# Autodesk Inventor assembly: KTN_MultiPass
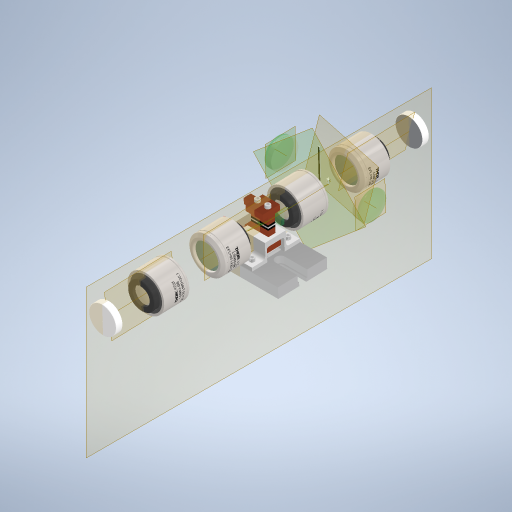
[picture p0: Inventor's stored thumbnail of the model, 512x512]
Saved by Autodesk Inventor 2023 (Build 270158000, 158)
## iProperties
Created: 2024-04-24
Part Number: KTN_MultiPass
Document SubType Name: Assembly
Designer: kerlin
Author: kerlin
## iProperties of the stored document base_Al_LEOD.ipt
Created: 2023-03-07
Part Number: bottomblock_al_ledgereod
Material: Aluminum 6061
Document SubType Name: Modeling
Designer: warke
Density: 2.7 g/cm^3
Appearance: Default
Sending System: Autodesk Inventor 2024
Author: warke
## iProperties of the stored document KTN_Chip_6p6mm_4mm_1p2mm_WithElectrodes.ipt
Created: 2022-10-15
Part Number: KTN_Chip_6p6mm_4mm_1p2mm_WithElectrodes
Material: Generic
Document SubType Name: Modeling
Designer: kerlin
Density: 1 g/cm^3
Appearance: Default
Sending System: Autodesk Inventor 2024
Author: kerlin
## iProperties of the stored document TEC3-2.5-Solidworks (1).ipt
Created: 2005-09-14
Part Number: TEC3-2.5-Solidworks (1)
Material: Generic
Document SubType Name: Modeling
Designer: warke
Density: 1 g/cm^3
Appearance: Default
Sending System: SolidWorks 2005
Last Author: rsavioli
Last Saved: 2005-09-14
Author: warke
## iProperties of the stored document 92196A107_18-8 Stainless Steel Socket Head Screw.ipt
Created: 2021-02-02
Part Number: 92196A107
Material: Generic
Description: 18-8 Stainless Steel Socket Head Screw
Vendor: McMaster-Carr Supply Company
Document SubType Name: Modeling
Designer: warke
Density: 1 g/cm^3
Appearance: Default
Sending System: SolidWorks 2017
Last Author: intuser33
Last Saved: 2023-02-03
Material: 18-8 Stainless Steel
Copyright: © 2023 McMaster-Carr Supply Company
CAD Model Disclaimer and Terms of Use: https://www.mcmaster.com/terms
Desc1: 18-8 Stainless Steel
Desc2: Socket Head Screw
Desc3: © 2023 McMaster-Carr Supply Company
Author: warke
## iProperties of the stored document spacer_AlN_LEOD.ipt
Created: 2023-03-13
Part Number: shapal_ledgereod
Material: Generic
Document SubType Name: Modeling
Designer: warke
Density: 1 g/cm^3
Appearance: Default
Sending System: Autodesk Inventor 2024
Author: warke
## iProperties of the stored document peltierclip_LEOD.ipt
Created: 2023-03-14
Part Number: peltierclip_ledgereod2
Material: Generic
Document SubType Name: Modeling
Designer: warke
Density: 1 g/cm^3
Appearance: Default
Sending System: Autodesk Inventor 2024
Author: warke
## iProperties of the stored document EOD_D1_v2.0.iam
Created: 2023-03-15
Part Number: EOD_D1_v2.0
Document SubType Name: Assembly
Designer: warke
Sending System: Autodesk Inventor 2024
Author: warke
## iProperties of the stored document 92949A105_18-8 Stainless Steel Button Head Hex Drive Screw.ipt
Created: 2019-06-06
Part Number: 92949A105_18-8 Stainless Steel Button Head Hex Drive Screw
Material: Stainless Steel, Austenitic
Description: 18-8 Stainless Steel Button Head Hex Drive Screw
Vendor: McMaster-Carr Supply Company
Document SubType Name: Modeling
Designer: warke
Density: 8 g/cm^3
Appearance: Default
Sending System: SolidWorks 2017
Last Author: intuser33
Last Saved: 2022-09-28
Material: 18-8 Stainless Steel
Copyright: © 2022 McMaster-Carr Supply Company
CAD Model Disclaimer and Terms of Use: https://www.mcmaster.com/terms
Desc1: 18-8 Stainless Steel Button
Desc2: Head Hex Drive Screw
Desc3: © 2022 McMaster-Carr Supply Company
Author: warke
## iProperties of the stored document electrode_Cu_LEOD.ipt
Created: 2023-03-13
Part Number: copper_top_ledgereod
Material: Copper
Document SubType Name: Modeling
Designer: warke
Density: 8.94 g/cm^3
Appearance: Default
Sending System: Autodesk Inventor 2024
Author: warke
## iProperties of the stored document graphite_LEOD.ipt
Created: 2023-03-13
Part Number: graphite_ledgereod
Material: Generic
Document SubType Name: Modeling
Designer: warke
Density: 1 g/cm^3
Appearance: Default
Sending System: Autodesk Inventor 2024
Author: warke
## iProperties of the stored document bottomblock_Cu_LEOD.ipt
Created: 2023-03-15
Part Number: bottom_cu_block
Material: Copper
Document SubType Name: Modeling
Designer: warke
Density: 8.94 g/cm^3
Appearance: Default
Sending System: Autodesk Inventor 2024
Author: warke
## iProperties of the stored document 95868A117_Nylon Socket Head Screws.ipt
Created: 2008-07-02
Part Number: 95868A117
Material: Generic
Description: Nylon Socket Head Screws
Vendor: McMaster-Carr Supply Company
Document SubType Name: Modeling
Designer: warke
Density: 1 g/cm^3
Appearance: Default
Sending System: SolidWorks 2017
Last Author: intuser33
Last Saved: 2021-07-09
Material: Nylon Plastic
Copyright: © 2021 McMaster-Carr Supply Company
CAD Model Disclaimer and Terms of Use: https://www.mcmaster.com/terms
Desc1: Nylon Socket
Desc2: Head Screws
Desc3: © 2021 McMaster-Carr Supply Company
Author: warke
## Documents named in this file (31)
- C:\Users\kerlin\Documents\KerlinLab\KTN\Multipass\MechanicalDrawing\KTN_MultiPass.iam
- C:\Users\kerlin\Documents\KerlinLab\KTN\Multipass\MechanicalDrawing\LSM03-BB-Solidworks.ipt
- C:\Users\kerlin\Documents\KerlinLab\KTN\Multipass\MechanicalDrawing\BB1-E02-Solidworks.ipt
- C:\Users\kerlin\Documents\KerlinLab\KTN\Multipass\MechanicalDrawing\MRA03-P01-Solidworks.ipt
- **C:\Users\kerlin\Documents\KerlinLab\KTN\Multipass\MechanicalDrawing\KTN_MultiPass.iam*LocalDocs*xAaaaasbaAaaaaaaaAaaaahvdAh*EOD_D1_v2.0.iam
- C:\Users\kerlin\Documents\KerlinLab\KTN\Multipass\MechanicalDrawing\ExitMirror.ipt
- C:\Users\kerlin\Documents\KerlinLab\KTN\Multipass\MechanicalDrawing\CylConcaveLens.ipt
- C:\Users\kerlin\Documents\KerlinLab\KTN\Multipass\MechanicalDrawing\Lens.ipt
- C:\Users\kerlin\Documents\KerlinLab\KTN\Multipass\MechanicalDrawing\pckngo_D1\EOD_D1_v2.0.iam
- C:\Users\kerlin\Documents\KerlinLab\KTN\Multipass\MechanicalDrawing\pckngo_D1\92196A107_18-8 Stainless Steel Socket Head Screw.ipt
- C:\Users\kerlin\Documents\KerlinLab\KTN\Multipass\MechanicalDrawing\pckngo_D1\92949A105_18-8 Stainless Steel Button Head Hex Drive Screw.ipt
- C:\Users\kerlin\Documents\KerlinLab\KTN\Multipass\MechanicalDrawing\pckngo_D1\95868A117_Nylon Socket Head Screws.ipt
- C:\Users\kerlin\Documents\KerlinLab\KTN\Multipass\MechanicalDrawing\pckngo_D1\base_Al_LEOD.ipt
- C:\Users\kerlin\Documents\KerlinLab\KTN\Multipass\MechanicalDrawing\pckngo_D1\bottomblock_Cu_LEOD.ipt
- C:\Users\kerlin\Documents\KerlinLab\KTN\Multipass\MechanicalDrawing\pckngo_D1\electrode_Cu_LEOD.ipt
- C:\Users\kerlin\Documents\KerlinLab\KTN\Multipass\MechanicalDrawing\pckngo_D1\graphite_LEOD.ipt
- C:\Users\kerlin\Documents\KerlinLab\KTN\Multipass\MechanicalDrawing\pckngo_D1\KTN_Chip_6p6mm_4mm_1p2mm_WithElectrodes.ipt
- C:\Users\kerlin\Documents\KerlinLab\KTN\Multipass\MechanicalDrawing\pckngo_D1\peltierclip_LEOD.ipt
- C:\Users\kerlin\Documents\KerlinLab\KTN\Multipass\MechanicalDrawing\pckngo_D1\spacer_AlN_LEOD.ipt
- C:\Users\kerlin\Documents\KerlinLab\KTN\Multipass\MechanicalDrawing\pckngo_D1\TEC3-2.5-Solidworks (1).ipt
- **C:\Users\kerlin\Documents\KerlinLab\KTN\Multipass\MechanicalDrawing\KTN_MultiPass.iam*LocalDocs*xAaaaapaaAaaaaaaaAaaaqtmnDd*base_Al_LEOD.ipt
- **C:\Users\kerlin\Documents\KerlinLab\KTN\Multipass\MechanicalDrawing\KTN_MultiPass.iam*LocalDocs*xAaaaadcaAaaaaaaaAaaaavr0Ea*KTN_Chip_6p6mm_4mm_1p2mm_WithElectrodes.ipt
- **C:\Users\kerlin\Documents\KerlinLab\KTN\Multipass\MechanicalDrawing\KTN_MultiPass.iam*LocalDocs*xAaaaadcaAaaaaaaaAaaaafrsWb*TEC3-2.5-Solidworks (1).ipt
- **C:\Users\kerlin\Documents\KerlinLab\KTN\Multipass\MechanicalDrawing\KTN_MultiPass.iam*LocalDocs*xAaaaaecaAaaaaaaaAaaaaqs5Gg*92196A107_18-8 Stainless Steel Socket Head Screw.ipt
- **C:\Users\kerlin\Documents\KerlinLab\KTN\Multipass\MechanicalDrawing\KTN_MultiPass.iam*LocalDocs*xAaaaqeaaAaaaaaaaAaaaqnhcGe*spacer_AlN_LEOD.ipt
- **C:\Users\kerlin\Documents\KerlinLab\KTN\Multipass\MechanicalDrawing\KTN_MultiPass.iam*LocalDocs*xAaaaatdaAaaaaaaaAaaaqlu4Jg*peltierclip_LEOD.ipt
- **C:\Users\kerlin\Documents\KerlinLab\KTN\Multipass\MechanicalDrawing\KTN_MultiPass.iam*LocalDocs*xAaaaqyaaAaaaaaaaAaaaaqtpDc*bottomblock_Cu_LEOD.ipt
- **C:\Users\kerlin\Documents\KerlinLab\KTN\Multipass\MechanicalDrawing\KTN_MultiPass.iam*LocalDocs*xAaaaqodaAaaaaaaaAaaaq2d30a*electrode_Cu_LEOD.ipt
- **C:\Users\kerlin\Documents\KerlinLab\KTN\Multipass\MechanicalDrawing\KTN_MultiPass.iam*LocalDocs*xAaaaqlcaAaaaaaaaAaaaalogYg*graphite_LEOD.ipt
- **C:\Users\kerlin\Documents\KerlinLab\KTN\Multipass\MechanicalDrawing\KTN_MultiPass.iam*LocalDocs*xAaaaq3baAaaaaaaaAaaaa4duMd*92949A105_18-8 Stainless Steel Button Head Hex Drive Screw.ipt
- **C:\Users\kerlin\Documents\KerlinLab\KTN\Multipass\MechanicalDrawing\KTN_MultiPass.iam*LocalDocs*xAaaaqzdaAaaaaaaaAaaaa3upGb*95868A117_Nylon Socket Head Screws.ipt
## Components (12 placed, 7 different names)
1. LSM03-BB-Solidworks:1 — Mate:3, Mate:4, Mate:5, Mate:6, Angle:2, Mate:13, Flush:6, Mate:14
2. LSM03-BB-Solidworks:2 — Mate:3, Mate:6, Mate:9, Mate:10
3. LSM03-BB-Solidworks:3 — Mate:1, Mate:7, Mate:8, Mate:11, Flush:4
4. LSM03-BB-Solidworks:4 — Mate:1, Mate:4, Mate:5, Mate:7, Flush:5
5. BB1-E02-Solidworks:1 — Mate:8, Mate:11, Mate:12
6. BB1-E02-Solidworks:2 — Mate:9, Mate:10
7. MRA03-P01-Solidworks:1 — Mate:12, Angle:1, Mate:14, Mate:15, Mate:16
8. EOD_D1_v2.0:1 [sub-assembly] — Flush:2
9. ExitMirror:1 — Angle:1
10. CylConcaveLens:1
11. Lens:1 — Mate:15
12. Lens:2 — Mate:16
## Relationships (21: Mate 15, Flush 4, Angle 2)
- Mate:1: LSM03-BB-Solidworks:3 ↔ LSM03-BB-Solidworks:4
- Mate:3: LSM03-BB-Solidworks:1 ↔ LSM03-BB-Solidworks:2
- Mate:4: LSM03-BB-Solidworks:1 ↔ LSM03-BB-Solidworks:4
- Mate:5 (40 mm): LSM03-BB-Solidworks:1 ↔ LSM03-BB-Solidworks:4
- Mate:6 (30 mm): LSM03-BB-Solidworks:1 ↔ LSM03-BB-Solidworks:2
- Mate:7 (30 mm): LSM03-BB-Solidworks:3 ↔ LSM03-BB-Solidworks:4
- Mate:8: LSM03-BB-Solidworks:3 ↔ BB1-E02-Solidworks:1
- Mate:9: LSM03-BB-Solidworks:2 ↔ BB1-E02-Solidworks:2
- Mate:10 (30 mm): LSM03-BB-Solidworks:2 ↔ BB1-E02-Solidworks:2
- Mate:11 (30 mm): LSM03-BB-Solidworks:3 ↔ BB1-E02-Solidworks:1
- Mate:12 (-82 mm): BB1-E02-Solidworks:1 ↔ MRA03-P01-Solidworks:1
- Angle:1 (0 deg): MRA03-P01-Solidworks:1 ↔ ExitMirror:1
- Angle:2 (0 deg): LSM03-BB-Solidworks:1
- Flush:2 (28 mm): EOD_D1_v2.0:1
- Mate:13: LSM03-BB-Solidworks:1
- Flush:4: LSM03-BB-Solidworks:3
- Flush:5: LSM03-BB-Solidworks:4
- Flush:6: LSM03-BB-Solidworks:1
- Mate:14: LSM03-BB-Solidworks:1 ↔ MRA03-P01-Solidworks:1
- Mate:15: MRA03-P01-Solidworks:1 ↔ Lens:1
- Mate:16: MRA03-P01-Solidworks:1 ↔ Lens:2
